# Autodesk Inventor assembly: kiteAssembly
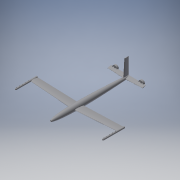
[picture p0: Inventor's stored thumbnail of the model, 180x180]
Saved by Autodesk Inventor 2019.3 (Build 233278000, 278)
## iProperties
Created: 2019-06-24
Part Number: kiteAssembly
Document SubType Name: Assembly
Designer: asiddiq2
Mass: 6.67535 g
Surface Area: 121.271 cm^2
Volume: 6.67535 cm^3
Density: 1 g/cm^3
Author: asiddiq2
## Documents named in this file (5)
- C:\Users\asiddiq2\Desktop\OCT_project\CAD_models\kite\kiteAssembly.iam
- C:\Users\asiddiq2\Desktop\OCT_project\CAD_models\kite\camberedWing.ipt
- C:\Users\asiddiq2\Desktop\OCT_project\CAD_models\kite\symmetricHS.ipt
- C:\Users\asiddiq2\Desktop\OCT_project\CAD_models\kite\symmetricVS.ipt
- C:\Users\asiddiq2\Desktop\OCT_project\CAD_models\kite\fuselage.ipt
## Components (4 placed, 4 different names)
1. camberedWing:1 — Flush:1, Flush:2, Flush:5, Flush:6, Flush:7, Flush:8
2. symmetricHS:1 — Flush:1, Flush:2, Flush:3, Mate:1, Flush:5, Flush:10, Flush:12
3. symmetricVS:1 — Flush:3, Mate:1, Flush:10
4. fuselage:1 — Mate:2, Mate:3, Flush:12
## Relationships (12: Flush 9, Mate 3)
- Flush:1: camberedWing:1 ↔ symmetricHS:1
- Flush:2: camberedWing:1 ↔ symmetricHS:1
- Flush:3: symmetricHS:1 ↔ symmetricVS:1
- Mate:1: symmetricHS:1 ↔ symmetricVS:1
- Flush:5 (90 mm): camberedWing:1 ↔ symmetricHS:1
- Flush:6: camberedWing:1
- Flush:7: camberedWing:1
- Flush:8: camberedWing:1
- Mate:2: fuselage:1
- Mate:3: fuselage:1
- Flush:10: symmetricHS:1 ↔ symmetricVS:1
- Flush:12 (-30 mm): symmetricHS:1 ↔ fuselage:1
## Named parameters: k_scale = 0.015, nom_chord = 15 mm, perc_HS_le = 6, HS_le = 90 mm
